# Autodesk Inventor assembly: E-AXIS ASSEMBLY P2.0
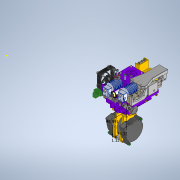
[picture p0: Inventor's stored thumbnail of the model, 180x180]
Saved by Autodesk Inventor 2020.3 (Build 243373010, 373A)
## iProperties
Created: 2019-12-19
Part Number: E-AXIS ASSEMBLY P2.0
Document SubType Name: Assembly
Designer: pepd9
Mass: 917.379 g
Surface Area: 2479.59 cm^2
Volume: 339.663 cm^3
Density: 2.70085 g/cm^3
Author: pepd9
## Documents named in this file (48)
- D:\Designs\MK3PRO P1\E-Axis\E-AXIS ASSEMBLY P2.0.iam
- D:\Designs\MK3PRO P1\E-Axis\X-Carriage V1.3.ipt
- D:\Designs\MK3PRO P1\COMPONENTS\M3 Nut.ipt
- D:\Designs\MK3PRO P1\COMPONENTS\NUT_SQUARE_M3.ipt
- D:\Designs\MK3PRO P1\COMPONENTS\LM10UU.ipt
- D:\Designs\MK3PRO P1\COMPONENTS\SHCS_M3_14.ipt
- D:\Designs\MK3PRO P1\E-Axis\Endstop Trigger Block.ipt
- D:\Designs\MK3PRO P1\COMPONENTS\SHCS_M3_20.ipt
- D:\Designs\MK3PRO P1\E-Axis\Extruder Back V2.ipt
- D:\Designs\MK3PRO P1\COMPONENTS\SHCS_M3_12.ipt
- D:\Designs\MK3PRO P1\E-Axis\Extruder Idler V2.ipt
- D:\Designs\MK3PRO P1\E-Axis\extruder-cover.ipt
- D:\Designs\MK3PRO P1\E-Axis\Fan Support Front.ipt
- D:\Designs\MK3PRO P1\E-Axis\Left Cable Guide.ipt
- D:\Designs\MK3PRO P1\COMPONENTS\SHCS_M3_35.ipt
- D:\Designs\MK3PRO P1\COMPONENTS\SHCS_M3_40.ipt
- D:\Designs\MK3PRO P1\COMPONENTS\Bondtech Idler.ipt
- D:\Designs\MK3PRO P1\E-Axis\PINDA_Probe.ipt
- D:\Designs\MK3PRO P1\E-Axis\E3D_V6.ipt
- D:\Designs\MK3PRO P1\E-Axis\E-Motor Mount P1.1.ipt
- D:\Designs\MK3PRO P1\E-Axis\Extruder_stepper_motor.iam
- D:\Designs\MK3PRO P1\COMPONENTS\SHCS_M3_8.ipt
- D:\Designs\MK3PRO P1\COMPONENTS\Bondtech Driver.ipt
- D:\Designs\MK3PRO P1\COMPONENTS\M3 Washer.ipt
- D:\Designs\MK3PRO P1\COMPONENTS\SHCS_M3_30.ipt
- D:\Designs\MK3PRO P1\COMPONENTS\FAN_5015_BLOWER.ipt
- D:\Designs\MK3PRO P1\COMPONENTS\SHCS_M3_25.ipt
- D:\Designs\MK3PRO P1\E-Axis\x-Carriage Backplate V1.2.ipt
- D:\Designs\MK3PRO P1\COMPONENTS\SHCS_M3_18.ipt
- D:\Designs\MK3PRO P1\E-Axis\LimitSwitch Container.ipt
- D:\Designs\MK3PRO P1\COMPONENTS\Noctua-NF-A4x10.ipt
- D:\Designs\MK3PRO P1\E-Axis\S Fan Cover.ipt
- D:\Designs\MK3PRO P1\COMPONENTS\Small Limit Switch.iam
- D:\Designs\MK3PRO P1\E-Axis\Extruder Cable Clamp.ipt
- D:\Designs\MK3PRO P1\E-Axis\Rear Fan Backplate Mount.ipt
- D:\Designs\MK3PRO P1\E-Axis\Rear Left Fan Mount.ipt
- D:\Designs\MK3PRO P1\E-Axis\Rear Right Fan Mount.ipt
- D:\Designs\MK3PRO P1\E-Axis\Rear Fan Spacer.ipt
- D:\Designs\MK3PRO P1\E2\Solenoid Assembly.iam
- D:\Designs\MK3PRO P1\E2\SolenoidBracket.ipt
- D:\Designs\MK3PRO P1\E2\TW-04-09.iam
- D:\Designs\MK3PRO P1\E2\TS-04-09-100.ipt
- D:\Designs\MK3PRO P1\COMPONENTS\SHCS_M2_10.ipt
- D:\Designs\MK3PRO P1\COMPONENTS\M2 Nut.ipt
- D:\Designs\MK3PRO P1\COMPONENTS\SHCS_M2x8.ipt
- D:\Designs\MK3PRO P1\E2\Slide.ipt
- D:\Designs\MK3PRO P1\E2\Link.ipt
- D:\Designs\MK3PRO P1\E2\extruder-coverE2.ipt
## Components (131 placed, 47 different names)
1. X-Carriage V1.3:1 — Flush:1, Mate:1, Mate:2, Mate:3, Mate:4, Mate:5, Mate:6, Mate:7, Mate:8, Mate:9, Mate:10, Mate:11, Mate:12, Mate:13, Mate:14, Mate:15, Mate:16, Mate:17, Mate:18, Mate:19, Mate:20, Angle:1, Angle:2, Angle:3, Angle:4, Angle:5, Angle:6, Angle:7, Angle:8, Angle:9, Mate:21, Mate:22, Angle:10, Mate:23, Mate:24, Mate:25, Mate:26, Mate:27, Mate:28, Mate:29, Mate:30, Mate:31, Mate:32, Mate:33, Mate:34, Angle:11, Mate:35, Mate:36, Angle:12, Mate:49, Mate:50, Mate:51, Mate:58, Mate:59, Mate:60, Mate:61, Mate:68, Mate:69, Mate:70, Mate:71, Mate:72, Mate:73, Mate:133, Mate:134, Mate:135, Mate:136, Mate:145, Mate:146, Mate:147
2. M3 Nut:1 — Mate:6, Mate:15, Angle:6
3. M3 Nut:2 — Mate:7, Mate:16, Angle:5
4. M3 Nut:3 — Mate:9, Mate:18, Angle:3
5. M3 Nut:4 — Mate:8, Mate:17, Angle:4
6. M3 Nut:5 — Mate:4, Mate:19, Angle:2
7. M3 Nut:6 — Mate:3, Mate:20, Angle:1
8. M3 Nut:7 — Mate:5, Mate:14, Angle:7
9. M3 Nut:8 — Mate:10, Mate:13, Angle:8
10. M3 Nut:9 — Mate:11, Mate:12, Angle:9
11. NUT_SQUARE_M3:1 — Mate:21, Mate:22, Angle:10
12. LM10UU:1 — Mate:25, Mate:28
13. LM10UU:2 — Mate:24, Mate:27
14. LM10UU:3 — Mate:23, Mate:26
15. SHCS_M3_14:1 — Mate:30, Mate:32
16. SHCS_M3_14:2 — Mate:29, Mate:31
17. Endstop Trigger Block:1 — Mate:35, Mate:36, Angle:12, Mate:37, Mate:38
18. NUT_SQUARE_M3:2 — Mate:33, Mate:34, Angle:11
19. SHCS_M3_20:1 — Mate:37, Mate:38
20. Extruder Back V2:1 — Mate:39, Mate:40, Mate:41, Mate:42, Mate:43, Mate:44, Mate:45, Mate:46, Angle:13, Mate:47, Angle:14, Mate:48, Angle:15, Mate:49, Mate:50, Mate:51, Mate:52, Mate:53, Angle:16, Mate:54, Mate:55, Mate:56, Mate:57, Angle:17, Angle:18, Mate:62, Mate:63, Angle:19, Mate:75, Mate:76, Mate:77, Mate:80, Mate:81, Angle:21, Mate:88, Mate:89, Mate:90, Flush:4, Mate:137, Mate:138, Angle:31, Angle:32, Mate:164, Mate:165, Angle:35, Mate:168, Mate:169, Mate:170, Mate:276, Angle:54, Mate:281, Mate:282, Flush:6, Mate:289, Mate:326, Mate:327, Mate:328, Mate:329, Angle:61, Angle:62, Mate:331, Mate:332, Mate:333
21. M3 Nut:10 — Mate:39, Mate:41
22. M3 Nut:11 — Mate:40, Mate:42
23. NUT_SQUARE_M3:3 — Mate:45, Mate:46, Angle:13
24. NUT_SQUARE_M3:4 — Mate:44, Mate:47, Angle:14
25. NUT_SQUARE_M3:5 — Mate:43, Mate:48, Angle:15
26. NUT_SQUARE_M3:6 — Mate:52, Mate:53, Angle:16
27. M3 Nut:12 — Mate:54, Mate:57, Angle:18
28. M3 Nut:13 — Mate:55, Mate:56, Angle:17
29. SHCS_M3_12:1 — Mate:58, Mate:60
30. SHCS_M3_12:2 — Mate:59, Mate:61
31. Extruder Idler V2:1 — Mate:74, Mate:75, Mate:78, Mate:79, Flush:4, Mate:92, Mate:93
32. extruder-cover:1 — Mate:96, Mate:97, Mate:98, Mate:99, Mate:100, Mate:101, Angle:24, Mate:102, Angle:25, Mate:103, Mate:104, Angle:26, Mate:105, Mate:106, Angle:27, Mate:107, Mate:108, Mate:109, Mate:110, Mate:111, Mate:112, Mate:113
33. Fan Support Front:1 — Mate:111, Mate:112, Mate:113, Mate:114, Mate:115, Mate:116, Mate:117, Mate:118, Mate:119, Angle:28, Mate:120, Mate:121, Angle:29, Mate:131, Mate:132, Mate:379, Mate:380
34. Left Cable Guide:1 — Mate:62, Mate:63, Angle:19, Mate:64, Mate:65, Angle:20, Mate:66, Mate:67, Mate:266, Mate:267, Angle:53, Mate:268, Mate:269, Mate:270
35. NUT_SQUARE_M3:7 — Mate:64, Mate:65, Angle:20
36. SHCS_M3_12:3 — Mate:66, Mate:67
37. SHCS_M3_35:1 — Mate:68, Mate:71, Mate:74
38. SHCS_M3_35:2 — Mate:70, Mate:73
39. SHCS_M3_35:3 — Mate:69, Mate:72
40. SHCS_M3_40:1 — Mate:76, Mate:77, Mate:94, Mate:95
41. Bondtech Idler:1 — Mate:78, Mate:79, Flush:3
42. PINDA_Probe:1 — Flush:2
43. E3D_V6:1 — Mate:80, Mate:81, Angle:21, Flush:2, Angle:63
44. E-Motor Mount P1.1:1 — Mate:83, Mate:84, Mate:85, Mate:86, Mate:87, Mate:88, Mate:89, Mate:90, Mate:96, Mate:97, Mate:98
45. Extruder_stepper_motor:1 [sub-assembly] — Mate:83, Mate:84, Mate:85, Mate:91
46. SHCS_M3_8:1 — Mate:86, Mate:87
47. Bondtech Driver:1 — Mate:91, Flush:3
48. M3 Washer:1 — Mate:92, Mate:93
49. M3 Washer:2 — Mate:94, Mate:95
50. NUT_SQUARE_M3:8 — Mate:105, Mate:106, Angle:27
51. NUT_SQUARE_M3:9 — Mate:103, Mate:104, Angle:26
52. NUT_SQUARE_M3:10 — Mate:100, Mate:101, Angle:24
53. NUT_SQUARE_M3:11 — Mate:99, Mate:102, Angle:25
54. SHCS_M3_30:1 — Mate:107, Mate:108
55. SHCS_M3_30:2 — Mate:109, Mate:110
56. M3 Nut:14 — Mate:118, Mate:119, Angle:28
57. M3 Nut:15 — Mate:120, Mate:121, Angle:29
58. SHCS_M3_8:2 — Mate:114, Mate:117
59. SHCS_M3_8:3 — Mate:115, Mate:116
60. SHCS_M3_20:2 — Mate:129, Mate:130, Mate:383
61. M3 Washer:3 — Mate:129, Mate:130, Mate:382
62. SHCS_M3_25:1 — Mate:131, Mate:132, Mate:381
63. SHCS_M3_12:4 — Mate:133, Mate:136, Mate:140
64. SHCS_M3_12:5 — Mate:134, Mate:135, Mate:139
65. M3 Nut:16 — Mate:137, Mate:140, Angle:32
66. M3 Nut:17 — Mate:138, Mate:139, Angle:31
67. x-Carriage Backplate V1.2:1 — Mate:141, Mate:142, Mate:143, Mate:144, Angle:33, Angle:34, Mate:145, Mate:146, Mate:147, Mate:148, Mate:149, Mate:150, Mate:151, Mate:152, Mate:153, Mate:154, Mate:155, Mate:156, Mate:157, Mate:158, Mate:159, Mate:160, Mate:161, Mate:162, Mate:163, Mate:187, Mate:214, Mate:275
68. M3 Nut:18 — Mate:141, Mate:144, Angle:33
69. M3 Nut:19 — Mate:142, Mate:143, Angle:34
70. SHCS_M3_18:1 — Mate:148, Mate:153
71. SHCS_M3_18:2 — Mate:149, Mate:151
72. SHCS_M3_18:3 — Mate:150, Mate:152
73. SHCS_M3_18:4 — Mate:154, Mate:155
74. SHCS_M3_18:5 — Mate:156, Mate:158
75. SHCS_M3_18:6 — Mate:157, Mate:159
76. SHCS_M3_18:7 — Mate:160, Mate:163
77. SHCS_M3_18:8 — Mate:161, Mate:162
78. LimitSwitch Container:1 — Mate:164, Mate:165, Angle:35, Mate:166, Mate:167, Mate:179, Mate:180, Mate:181
79. SHCS_M3_8:4 — Mate:166, Mate:167
80. Noctua-NF-A4x10:1 — Mate:168, Mate:169, Mate:170, Mate:171, Mate:172, Mate:173, Mate:174, Mate:248
81. SHCS_M3_18:9 — Mate:172, Mate:249
82. SHCS_M3_18:10 — Mate:171
83. SHCS_M3_18:11 — Mate:173, Mate:250
84. SHCS_M3_18:12 — Mate:174
85. Small Limit Switch:1 [sub-assembly] — Mate:179, Mate:180, Mate:181
86. Rear Fan Backplate Mount:1 — Mate:182, Mate:183, Mate:184, Mate:185, Angle:37, Mate:187, Mate:188, Mate:189, Mate:190, Mate:191, Mate:200, Mate:201, Mate:202, Mate:203, Angle:52, Mate:275
87. M3 Nut:20 — Mate:182, Mate:184
88. M3 Nut:21 — Mate:183, Mate:185, Angle:37
89. SHCS_M3_12:6 — Mate:188, Mate:189
90. SHCS_M3_14:3 — Mate:190, Mate:191, Mate:214
91. Rear Left Fan Mount:1 — Mate:198, Angle:40, Mate:201, Mate:202, Mate:205, Mate:206, Mate:207, Mate:219, Mate:222, Angle:52, Mate:374, Angle:66
92. Rear Right Fan Mount:1 — Mate:196, Angle:42, Mate:200, Mate:203, Mate:204, Mate:208, Mate:209, Mate:220, Mate:221, Mate:373, Angle:65, Mate:377
93. M3 Nut:22 — Mate:196, Angle:42, Mate:265
94. M3 Nut:25 — Mate:198, Angle:40, Mate:246
95. FAN_5015_BLOWER:2 — Mate:204, Mate:208, Mate:209, Mate:242, Mate:243, Mate:255, Mate:256
96. FAN_5015_BLOWER:3 — Mate:205, Mate:206, Mate:207, Mate:240, Mate:241, Mate:371, Mate:372
97. SHCS_M3_14:4 — Mate:219, Mate:222
98. SHCS_M3_14:5 — Mate:220, Mate:221
99. SHCS_M3_25:2 — Mate:240, Mate:241, Mate:247
100. SHCS_M3_25:3 — Mate:242, Mate:244, Mate:245
101. M3 Washer:4 — Mate:243, Mate:244, Mate:245
102. Rear Fan Spacer:1 — Mate:246, Mate:247, Mate:265
103. S Fan Cover:1 — Mate:248, Mate:249, Mate:250
104. SHCS_M3_18:13 — Mate:271, Mate:274
105. SHCS_M3_25:4 — Mate:255, Mate:257, Mate:258, Mate:376, Mate:378
106. M3 Washer:5 — Mate:256, Mate:257, Mate:258
107. NUT_SQUARE_M3:12 — Mate:266, Mate:267, Angle:53
108. SHCS_M3_18:14 — Mate:272, Mate:273
109. Extruder Cable Clamp:1 — Mate:268, Mate:269, Mate:270, Mate:271, Mate:272, Mate:273, Mate:274
110. Solenoid Assembly:1 [sub-assembly] — Mate:276, Angle:54, Mate:278, Mate:280
111. SolenoidBracket:1 — Mate:278, Mate:280, Mate:281, Mate:282
112. TW-04-09:1 [sub-assembly] — Mate:290, Mate:300, Mate:341, Mate:342, Mate:361
113. TS-04-09-100:1 — Mate:289, Mate:290, Flush:6, Mate:300
114. SHCS_M2_10:1 — Flush:15
115. SHCS_M2_10:3 — Flush:13, Mate:342, Mate:362
116. SHCS_M2_10:4 — Flush:13, Flush:14, Flush:15
117. M2 Nut:1 — Mate:326, Mate:329, Angle:61
118. M2 Nut:2 — Mate:327, Mate:328, Angle:62
119. SHCS_M2x8:2 — Mate:331, Flush:12
120. SHCS_M2x8:3 — Mate:332, Mate:333, Flush:12
121. SHCS_M2_10:5 — Flush:14, Mate:341, Mate:363
122. extruder-coverE2:1 — Mate:365, Angle:64, Mate:367
123. Link:1 — Mate:358, Mate:359, Mate:360
124. Slide:1 — Mate:358, Mate:359, Mate:360, Mate:361, Mate:362, Mate:363, Mate:364, Flush:16, Angle:64, Mate:368, Mate:369, Mate:370
125. E3D_V6:2 — Mate:364, Flush:16, Angle:63, Mate:365
126. Noctua-NF-A4x10:2 — Mate:367, Mate:368, Mate:369, Mate:370
127. SHCS_M3_25:5 — Mate:371, Mate:372, Mate:375
128. M3 Nut:26 — Mate:373, Mate:376, Angle:65
129. M3 Nut:27 — Mate:374, Mate:375, Angle:66
130. Rear Fan Spacer:2 — Mate:377, Mate:378
131. FAN_5015_BLOWER:4 — Mate:379, Mate:380, Mate:381, Mate:382, Mate:383
## Relationships (317: Mate 263, Angle 44, Flush 10)
- Flush:1: X-Carriage V1.3:1
- Mate:1 (8.3 mm): X-Carriage V1.3:1
- Mate:2 (-43.75 mm): X-Carriage V1.3:1
- Mate:3: X-Carriage V1.3:1 ↔ M3 Nut:6
- Mate:4: X-Carriage V1.3:1 ↔ M3 Nut:5
- Mate:5: X-Carriage V1.3:1 ↔ M3 Nut:7
- Mate:6: X-Carriage V1.3:1 ↔ M3 Nut:1
- Mate:7: X-Carriage V1.3:1 ↔ M3 Nut:2
- Mate:8: X-Carriage V1.3:1 ↔ M3 Nut:4
- Mate:9: X-Carriage V1.3:1 ↔ M3 Nut:3
- Mate:10: X-Carriage V1.3:1 ↔ M3 Nut:8
- Mate:11: X-Carriage V1.3:1 ↔ M3 Nut:9
- Mate:12: X-Carriage V1.3:1 ↔ M3 Nut:9
- Mate:13: X-Carriage V1.3:1 ↔ M3 Nut:8
- Mate:14: X-Carriage V1.3:1 ↔ M3 Nut:7
- Mate:15: X-Carriage V1.3:1 ↔ M3 Nut:1
- Mate:16: X-Carriage V1.3:1 ↔ M3 Nut:2
- Mate:17: X-Carriage V1.3:1 ↔ M3 Nut:4
- Mate:18: X-Carriage V1.3:1 ↔ M3 Nut:3
- Mate:19: X-Carriage V1.3:1 ↔ M3 Nut:5
- Mate:20: X-Carriage V1.3:1 ↔ M3 Nut:6
- Angle:1 (0 deg): X-Carriage V1.3:1 ↔ M3 Nut:6
- Angle:2 (0 deg): X-Carriage V1.3:1 ↔ M3 Nut:5
- Angle:3 (0 deg): X-Carriage V1.3:1 ↔ M3 Nut:3
- Angle:4 (0 deg): X-Carriage V1.3:1 ↔ M3 Nut:4
- Angle:5 (0 deg): X-Carriage V1.3:1 ↔ M3 Nut:2
- Angle:6 (0 deg): X-Carriage V1.3:1 ↔ M3 Nut:1
- Angle:7 (0 deg): X-Carriage V1.3:1 ↔ M3 Nut:7
- Angle:8 (0 deg): X-Carriage V1.3:1 ↔ M3 Nut:8
- Angle:9 (0 deg): X-Carriage V1.3:1 ↔ M3 Nut:9
- Mate:21: X-Carriage V1.3:1 ↔ NUT_SQUARE_M3:1
- Mate:22: X-Carriage V1.3:1 ↔ NUT_SQUARE_M3:1
- Angle:10 (0 deg): X-Carriage V1.3:1 ↔ NUT_SQUARE_M3:1
- Mate:23: X-Carriage V1.3:1 ↔ LM10UU:3
- Mate:24: X-Carriage V1.3:1 ↔ LM10UU:2
- Mate:25: X-Carriage V1.3:1 ↔ LM10UU:1
- Mate:26 (0.25 mm): X-Carriage V1.3:1 ↔ LM10UU:3
- Mate:27 (0.25 mm): X-Carriage V1.3:1 ↔ LM10UU:2
- Mate:28 (0.25 mm): X-Carriage V1.3:1 ↔ LM10UU:1
- Mate:29: X-Carriage V1.3:1 ↔ SHCS_M3_14:2
- Mate:30: X-Carriage V1.3:1 ↔ SHCS_M3_14:1
- Mate:31: X-Carriage V1.3:1 ↔ SHCS_M3_14:2
- Mate:32: X-Carriage V1.3:1 ↔ SHCS_M3_14:1
- Mate:33: X-Carriage V1.3:1 ↔ NUT_SQUARE_M3:2
- Mate:34: X-Carriage V1.3:1 ↔ NUT_SQUARE_M3:2
- Angle:11 (0 deg): X-Carriage V1.3:1 ↔ NUT_SQUARE_M3:2
- Mate:35: X-Carriage V1.3:1 ↔ Endstop Trigger Block:1
- Mate:36: X-Carriage V1.3:1 ↔ Endstop Trigger Block:1
- Angle:12 (180 deg): X-Carriage V1.3:1 ↔ Endstop Trigger Block:1
- Mate:37: Endstop Trigger Block:1 ↔ SHCS_M3_20:1
- Mate:38: Endstop Trigger Block:1 ↔ SHCS_M3_20:1
- Mate:39: Extruder Back V2:1 ↔ M3 Nut:10
- Mate:40: Extruder Back V2:1 ↔ M3 Nut:11
- Mate:41: Extruder Back V2:1 ↔ M3 Nut:10
- Mate:42: Extruder Back V2:1 ↔ M3 Nut:11
- Mate:43: Extruder Back V2:1 ↔ NUT_SQUARE_M3:5
- Mate:44: Extruder Back V2:1 ↔ NUT_SQUARE_M3:4
- Mate:45: Extruder Back V2:1 ↔ NUT_SQUARE_M3:3
- Mate:46: Extruder Back V2:1 ↔ NUT_SQUARE_M3:3
- Angle:13 (0 deg): Extruder Back V2:1 ↔ NUT_SQUARE_M3:3
- Mate:47: Extruder Back V2:1 ↔ NUT_SQUARE_M3:4
- Angle:14 (0 deg): Extruder Back V2:1 ↔ NUT_SQUARE_M3:4
- Mate:48: Extruder Back V2:1 ↔ NUT_SQUARE_M3:5
- Angle:15 (0 deg): Extruder Back V2:1 ↔ NUT_SQUARE_M3:5
- Mate:49: X-Carriage V1.3:1 ↔ Extruder Back V2:1
- Mate:50: X-Carriage V1.3:1 ↔ Extruder Back V2:1
- Mate:51: X-Carriage V1.3:1 ↔ Extruder Back V2:1
- Mate:52: Extruder Back V2:1 ↔ NUT_SQUARE_M3:6
- Mate:53: Extruder Back V2:1 ↔ NUT_SQUARE_M3:6
- Angle:16 (0 deg): Extruder Back V2:1 ↔ NUT_SQUARE_M3:6
- Mate:54: Extruder Back V2:1 ↔ M3 Nut:12
- Mate:55: Extruder Back V2:1 ↔ M3 Nut:13
- Mate:56: Extruder Back V2:1 ↔ M3 Nut:13
- Mate:57: Extruder Back V2:1 ↔ M3 Nut:12
- Angle:17 (0 deg): Extruder Back V2:1 ↔ M3 Nut:13
- Angle:18 (0 deg): Extruder Back V2:1 ↔ M3 Nut:12
- Mate:58: X-Carriage V1.3:1 ↔ SHCS_M3_12:1
- Mate:59: X-Carriage V1.3:1 ↔ SHCS_M3_12:2
- Mate:60: X-Carriage V1.3:1 ↔ SHCS_M3_12:1
- Mate:61: X-Carriage V1.3:1 ↔ SHCS_M3_12:2
- Mate:62: Extruder Back V2:1 ↔ Left Cable Guide:1
- Mate:63: Extruder Back V2:1 ↔ Left Cable Guide:1
- Angle:19 (180 deg): Extruder Back V2:1 ↔ Left Cable Guide:1
- Mate:64: Left Cable Guide:1 ↔ NUT_SQUARE_M3:7
- Mate:65: Left Cable Guide:1 ↔ NUT_SQUARE_M3:7
- Angle:20 (0 deg): Left Cable Guide:1 ↔ NUT_SQUARE_M3:7
- Mate:66: Left Cable Guide:1 ↔ SHCS_M3_12:3
- Mate:67: Left Cable Guide:1 ↔ SHCS_M3_12:3
- Mate:68: X-Carriage V1.3:1 ↔ SHCS_M3_35:1
- Mate:69: X-Carriage V1.3:1 ↔ SHCS_M3_35:3
- Mate:70: X-Carriage V1.3:1 ↔ SHCS_M3_35:2
- Mate:71: X-Carriage V1.3:1 ↔ SHCS_M3_35:1
- Mate:72: X-Carriage V1.3:1 ↔ SHCS_M3_35:3
- Mate:73: X-Carriage V1.3:1 ↔ SHCS_M3_35:2
- Mate:74: Extruder Idler V2:1 ↔ SHCS_M3_35:1
- Mate:75 (0.5 mm): Extruder Back V2:1 ↔ Extruder Idler V2:1
- Mate:76: Extruder Back V2:1 ↔ SHCS_M3_40:1
- Mate:77: Extruder Back V2:1 ↔ SHCS_M3_40:1
- Mate:78: Extruder Idler V2:1 ↔ Bondtech Idler:1
- Mate:79 (0.25 mm): Extruder Idler V2:1 ↔ Bondtech Idler:1
- Mate:80: Extruder Back V2:1 ↔ E3D_V6:1
- Mate:81: Extruder Back V2:1 ↔ E3D_V6:1
- Angle:21 (90 deg): Extruder Back V2:1 ↔ E3D_V6:1
- Flush:2 (2 mm): PINDA_Probe:1 ↔ E3D_V6:1
- Mate:83: E-Motor Mount P1.1:1 ↔ Extruder_stepper_motor:1
- Mate:84: E-Motor Mount P1.1:1 ↔ Extruder_stepper_motor:1
- Mate:85: E-Motor Mount P1.1:1 ↔ Extruder_stepper_motor:1
- Mate:86: E-Motor Mount P1.1:1 ↔ SHCS_M3_8:1
- Mate:87: E-Motor Mount P1.1:1 ↔ SHCS_M3_8:1
- Mate:88: Extruder Back V2:1 ↔ E-Motor Mount P1.1:1
- Mate:89: Extruder Back V2:1 ↔ E-Motor Mount P1.1:1
- Mate:90: Extruder Back V2:1 ↔ E-Motor Mount P1.1:1
- Mate:91: Extruder_stepper_motor:1 ↔ Bondtech Driver:1
- Flush:3: Bondtech Idler:1 ↔ Bondtech Driver:1
- Flush:4: Extruder Back V2:1 ↔ Extruder Idler V2:1
- Mate:92: Extruder Idler V2:1 ↔ M3 Washer:1
- Mate:93: Extruder Idler V2:1 ↔ M3 Washer:1
- Mate:94: SHCS_M3_40:1 ↔ M3 Washer:2
- Mate:95: SHCS_M3_40:1 ↔ M3 Washer:2
- Mate:96: extruder-cover:1 ↔ E-Motor Mount P1.1:1
- Mate:97: extruder-cover:1 ↔ E-Motor Mount P1.1:1
- Mate:98: extruder-cover:1 ↔ E-Motor Mount P1.1:1
- Mate:99: extruder-cover:1 ↔ NUT_SQUARE_M3:11
- Mate:100: extruder-cover:1 ↔ NUT_SQUARE_M3:10
- Mate:101: extruder-cover:1 ↔ NUT_SQUARE_M3:10
- Angle:24 (0 deg): extruder-cover:1 ↔ NUT_SQUARE_M3:10
- Mate:102: extruder-cover:1 ↔ NUT_SQUARE_M3:11
- Angle:25 (0 deg): extruder-cover:1 ↔ NUT_SQUARE_M3:11
- Mate:103: extruder-cover:1 ↔ NUT_SQUARE_M3:9
- Mate:104: extruder-cover:1 ↔ NUT_SQUARE_M3:9
- Angle:26 (0 deg): extruder-cover:1 ↔ NUT_SQUARE_M3:9
- Mate:105: extruder-cover:1 ↔ NUT_SQUARE_M3:8
- Mate:106: extruder-cover:1 ↔ NUT_SQUARE_M3:8
- Angle:27 (0 deg): extruder-cover:1 ↔ NUT_SQUARE_M3:8
- Mate:107: extruder-cover:1 ↔ SHCS_M3_30:1
- Mate:108: extruder-cover:1 ↔ SHCS_M3_30:1
- Mate:109: extruder-cover:1 ↔ SHCS_M3_30:2
- Mate:110: extruder-cover:1 ↔ SHCS_M3_30:2
- Mate:111: extruder-cover:1 ↔ Fan Support Front:1
- Mate:112: extruder-cover:1 ↔ Fan Support Front:1
- Mate:113: extruder-cover:1 ↔ Fan Support Front:1
- Mate:114: Fan Support Front:1 ↔ SHCS_M3_8:2
- Mate:115: Fan Support Front:1 ↔ SHCS_M3_8:3
- Mate:116: Fan Support Front:1 ↔ SHCS_M3_8:3
- Mate:117: Fan Support Front:1 ↔ SHCS_M3_8:2
- Mate:118: Fan Support Front:1 ↔ M3 Nut:14
- Mate:119: Fan Support Front:1 ↔ M3 Nut:14
- Angle:28 (0 deg): Fan Support Front:1 ↔ M3 Nut:14
- Mate:120: Fan Support Front:1 ↔ M3 Nut:15
- Mate:121: Fan Support Front:1 ↔ M3 Nut:15
- Angle:29 (30 deg): Fan Support Front:1 ↔ M3 Nut:15
- Mate:129: SHCS_M3_20:2 ↔ M3 Washer:3
- Mate:130: SHCS_M3_20:2 ↔ M3 Washer:3
- Mate:131: Fan Support Front:1 ↔ SHCS_M3_25:1
- Mate:132: Fan Support Front:1 ↔ SHCS_M3_25:1
- Mate:133: X-Carriage V1.3:1 ↔ SHCS_M3_12:4
- Mate:134: X-Carriage V1.3:1 ↔ SHCS_M3_12:5
- Mate:135: X-Carriage V1.3:1 ↔ SHCS_M3_12:5
- Mate:136: X-Carriage V1.3:1 ↔ SHCS_M3_12:4
- Mate:137: Extruder Back V2:1 ↔ M3 Nut:16
- Mate:138: Extruder Back V2:1 ↔ M3 Nut:17
- Mate:139: SHCS_M3_12:5 ↔ M3 Nut:17
- Angle:31 (0 deg): Extruder Back V2:1 ↔ M3 Nut:17
- Mate:140: SHCS_M3_12:4 ↔ M3 Nut:16
- Angle:32 (0 deg): Extruder Back V2:1 ↔ M3 Nut:16
- Mate:141: x-Carriage Backplate V1.2:1 ↔ M3 Nut:18
- Mate:142: x-Carriage Backplate V1.2:1 ↔ M3 Nut:19
- Mate:143: x-Carriage Backplate V1.2:1 ↔ M3 Nut:19
- Mate:144: x-Carriage Backplate V1.2:1 ↔ M3 Nut:18
- Angle:33 (0 deg): x-Carriage Backplate V1.2:1 ↔ M3 Nut:18
- Angle:34 (0 deg): x-Carriage Backplate V1.2:1 ↔ M3 Nut:19
- Mate:145: X-Carriage V1.3:1 ↔ x-Carriage Backplate V1.2:1
- Mate:146: X-Carriage V1.3:1 ↔ x-Carriage Backplate V1.2:1
- Mate:147: X-Carriage V1.3:1 ↔ x-Carriage Backplate V1.2:1
- Mate:148: x-Carriage Backplate V1.2:1 ↔ SHCS_M3_18:1
- Mate:149: x-Carriage Backplate V1.2:1 ↔ SHCS_M3_18:2
- Mate:150: x-Carriage Backplate V1.2:1 ↔ SHCS_M3_18:3
- Mate:151: x-Carriage Backplate V1.2:1 ↔ SHCS_M3_18:2
- Mate:152: x-Carriage Backplate V1.2:1 ↔ SHCS_M3_18:3
- Mate:153: x-Carriage Backplate V1.2:1 ↔ SHCS_M3_18:1
- Mate:154: x-Carriage Backplate V1.2:1 ↔ SHCS_M3_18:4
- Mate:155: x-Carriage Backplate V1.2:1 ↔ SHCS_M3_18:4
- Mate:156: x-Carriage Backplate V1.2:1 ↔ SHCS_M3_18:5
- Mate:157: x-Carriage Backplate V1.2:1 ↔ SHCS_M3_18:6
- Mate:158: x-Carriage Backplate V1.2:1 ↔ SHCS_M3_18:5
- Mate:159: x-Carriage Backplate V1.2:1 ↔ SHCS_M3_18:6
- Mate:160: x-Carriage Backplate V1.2:1 ↔ SHCS_M3_18:7
- Mate:161: x-Carriage Backplate V1.2:1 ↔ SHCS_M3_18:8
- Mate:162: x-Carriage Backplate V1.2:1 ↔ SHCS_M3_18:8
- Mate:163: x-Carriage Backplate V1.2:1 ↔ SHCS_M3_18:7
- Mate:164: Extruder Back V2:1 ↔ LimitSwitch Container:1
- Mate:165: Extruder Back V2:1 ↔ LimitSwitch Container:1
- Angle:35 (180 deg): Extruder Back V2:1 ↔ LimitSwitch Container:1
- Mate:166: LimitSwitch Container:1 ↔ SHCS_M3_8:4
- Mate:167: LimitSwitch Container:1 ↔ SHCS_M3_8:4
- Mate:168: Extruder Back V2:1 ↔ Noctua-NF-A4x10:1
- Mate:169: Extruder Back V2:1 ↔ Noctua-NF-A4x10:1
- Mate:170: Extruder Back V2:1 ↔ Noctua-NF-A4x10:1
- Mate:171: Noctua-NF-A4x10:1 ↔ SHCS_M3_18:10
- Mate:172: Noctua-NF-A4x10:1 ↔ SHCS_M3_18:9
- Mate:173: Noctua-NF-A4x10:1 ↔ SHCS_M3_18:11
- Mate:174: Noctua-NF-A4x10:1 ↔ SHCS_M3_18:12
- Mate:179: LimitSwitch Container:1 ↔ Small Limit Switch:1
- Mate:180: LimitSwitch Container:1 ↔ Small Limit Switch:1
- Mate:181: LimitSwitch Container:1 ↔ Small Limit Switch:1
- Mate:182: Rear Fan Backplate Mount:1 ↔ M3 Nut:20
- Mate:183: Rear Fan Backplate Mount:1 ↔ M3 Nut:21
- Mate:184: Rear Fan Backplate Mount:1 ↔ M3 Nut:20
- Mate:185: Rear Fan Backplate Mount:1 ↔ M3 Nut:21
- Angle:37 (0 deg): Rear Fan Backplate Mount:1 ↔ M3 Nut:21
- Mate:187: x-Carriage Backplate V1.2:1 ↔ Rear Fan Backplate Mount:1
- Mate:188: Rear Fan Backplate Mount:1 ↔ SHCS_M3_12:6
- Mate:189: Rear Fan Backplate Mount:1 ↔ SHCS_M3_12:6
- Mate:190: Rear Fan Backplate Mount:1 ↔ SHCS_M3_14:3
- Mate:191: Rear Fan Backplate Mount:1 ↔ SHCS_M3_14:3
- Mate:196: Rear Right Fan Mount:1 ↔ M3 Nut:22
- Mate:198: Rear Left Fan Mount:1 ↔ M3 Nut:25
- Angle:40 (0 deg): Rear Left Fan Mount:1 ↔ M3 Nut:25
- Angle:42 (0 deg): Rear Right Fan Mount:1 ↔ M3 Nut:22
- Mate:200: Rear Fan Backplate Mount:1 ↔ Rear Right Fan Mount:1
- Mate:201: Rear Fan Backplate Mount:1 ↔ Rear Left Fan Mount:1
- Mate:202: Rear Fan Backplate Mount:1 ↔ Rear Left Fan Mount:1
- Mate:203: Rear Fan Backplate Mount:1 ↔ Rear Right Fan Mount:1
- Mate:204: Rear Right Fan Mount:1 ↔ FAN_5015_BLOWER:2
- Mate:205: Rear Left Fan Mount:1 ↔ FAN_5015_BLOWER:3
- Mate:206: Rear Left Fan Mount:1 ↔ FAN_5015_BLOWER:3
- Mate:207: Rear Left Fan Mount:1 ↔ FAN_5015_BLOWER:3
- Mate:208: Rear Right Fan Mount:1 ↔ FAN_5015_BLOWER:2
- Mate:209: Rear Right Fan Mount:1 ↔ FAN_5015_BLOWER:2
- Mate:214: x-Carriage Backplate V1.2:1 ↔ SHCS_M3_14:3
- Mate:219: Rear Left Fan Mount:1 ↔ SHCS_M3_14:4
- Mate:220: Rear Right Fan Mount:1 ↔ SHCS_M3_14:5
- Mate:221: Rear Right Fan Mount:1 ↔ SHCS_M3_14:5
- Mate:222: Rear Left Fan Mount:1 ↔ SHCS_M3_14:4
- Mate:240: FAN_5015_BLOWER:3 ↔ SHCS_M3_25:2
- Mate:241: FAN_5015_BLOWER:3 ↔ SHCS_M3_25:2
- Mate:242: FAN_5015_BLOWER:2 ↔ SHCS_M3_25:3
- Mate:243: FAN_5015_BLOWER:2 ↔ M3 Washer:4
- Mate:244: SHCS_M3_25:3 ↔ M3 Washer:4
- Mate:245: SHCS_M3_25:3 ↔ M3 Washer:4
- Mate:246: M3 Nut:25 ↔ Rear Fan Spacer:1
- Mate:247: SHCS_M3_25:2 ↔ Rear Fan Spacer:1
- Mate:248: Noctua-NF-A4x10:1 ↔ S Fan Cover:1
- Mate:249: SHCS_M3_18:9 ↔ S Fan Cover:1
- Mate:250: SHCS_M3_18:11 ↔ S Fan Cover:1
- Mate:255: FAN_5015_BLOWER:2 ↔ SHCS_M3_25:4
- Mate:256: FAN_5015_BLOWER:2 ↔ M3 Washer:5
- Mate:257: SHCS_M3_25:4 ↔ M3 Washer:5
- Mate:258: SHCS_M3_25:4 ↔ M3 Washer:5
- Mate:265: M3 Nut:22 ↔ Rear Fan Spacer:1
- Angle:52 (0 deg): Rear Fan Backplate Mount:1 ↔ Rear Left Fan Mount:1
- Mate:266: Left Cable Guide:1 ↔ NUT_SQUARE_M3:12
- Mate:267: Left Cable Guide:1 ↔ NUT_SQUARE_M3:12
- Angle:53 (0 deg): Left Cable Guide:1 ↔ NUT_SQUARE_M3:12
- Mate:268: Left Cable Guide:1 ↔ Extruder Cable Clamp:1
- Mate:269: Left Cable Guide:1 ↔ Extruder Cable Clamp:1
- Mate:270: Left Cable Guide:1 ↔ Extruder Cable Clamp:1
- Mate:271: SHCS_M3_18:13 ↔ Extruder Cable Clamp:1
- Mate:272: SHCS_M3_18:14 ↔ Extruder Cable Clamp:1
- Mate:273: SHCS_M3_18:14 ↔ Extruder Cable Clamp:1
- Mate:274: SHCS_M3_18:13 ↔ Extruder Cable Clamp:1
- Mate:275: x-Carriage Backplate V1.2:1 ↔ Rear Fan Backplate Mount:1
- Mate:276: Extruder Back V2:1 ↔ Solenoid Assembly:1
- Angle:54 (0 deg): Extruder Back V2:1 ↔ Solenoid Assembly:1
- Mate:278: Solenoid Assembly:1 ↔ SolenoidBracket:1
- Mate:280: Solenoid Assembly:1 ↔ SolenoidBracket:1
- Mate:281: Extruder Back V2:1 ↔ SolenoidBracket:1
- Mate:282: Extruder Back V2:1 ↔ SolenoidBracket:1
- Mate:289: Extruder Back V2:1 ↔ TS-04-09-100:1
- Mate:290: TW-04-09:1 ↔ TS-04-09-100:1
- Flush:6: Extruder Back V2:1 ↔ TS-04-09-100:1
- Mate:300: TW-04-09:1 ↔ TS-04-09-100:1
- Mate:326: Extruder Back V2:1 ↔ M2 Nut:1
- Mate:327: Extruder Back V2:1 ↔ M2 Nut:2
- Mate:328: Extruder Back V2:1 ↔ M2 Nut:2
- Mate:329: Extruder Back V2:1 ↔ M2 Nut:1
- Angle:61 (0 deg): Extruder Back V2:1 ↔ M2 Nut:1
- Angle:62 (0 deg): Extruder Back V2:1 ↔ M2 Nut:2
- Mate:331: Extruder Back V2:1 ↔ SHCS_M2x8:2
- Mate:332: Extruder Back V2:1 ↔ SHCS_M2x8:3
- Mate:333 (4.6 mm): Extruder Back V2:1 ↔ SHCS_M2x8:3
- Flush:12: SHCS_M2x8:2 ↔ SHCS_M2x8:3
- Flush:13: SHCS_M2_10:3 ↔ SHCS_M2_10:4
- Flush:14: SHCS_M2_10:4 ↔ SHCS_M2_10:5
- Flush:15: SHCS_M2_10:1 ↔ SHCS_M2_10:4
- Mate:341: TW-04-09:1 ↔ SHCS_M2_10:5
- Mate:342: TW-04-09:1 ↔ SHCS_M2_10:3
- Mate:358: Link:1 ↔ Slide:1
- Mate:359: Link:1 ↔ Slide:1
- Mate:360: Link:1 ↔ Slide:1
- Mate:361: TW-04-09:1 ↔ Slide:1
- Mate:362: SHCS_M2_10:3 ↔ Slide:1
- Mate:363: SHCS_M2_10:5 ↔ Slide:1
- Mate:364: Slide:1 ↔ E3D_V6:2
- Flush:16: Slide:1 ↔ E3D_V6:2
- Angle:63 (0 deg): E3D_V6:1 ↔ E3D_V6:2
- Mate:365: extruder-coverE2:1 ↔ E3D_V6:2
- Angle:64 (0 deg): extruder-coverE2:1 ↔ Slide:1
- Mate:367: extruder-coverE2:1 ↔ Noctua-NF-A4x10:2
- Mate:368: Slide:1 ↔ Noctua-NF-A4x10:2
- Mate:369: Slide:1 ↔ Noctua-NF-A4x10:2
- Mate:370: Slide:1 ↔ Noctua-NF-A4x10:2
- Mate:371: FAN_5015_BLOWER:3 ↔ SHCS_M3_25:5
- Mate:372: FAN_5015_BLOWER:3 ↔ SHCS_M3_25:5
- Mate:373: Rear Right Fan Mount:1 ↔ M3 Nut:26
- Mate:374: Rear Left Fan Mount:1 ↔ M3 Nut:27
- Mate:375: SHCS_M3_25:5 ↔ M3 Nut:27
- Mate:376: SHCS_M3_25:4 ↔ M3 Nut:26
- Angle:65 (0 deg): Rear Right Fan Mount:1 ↔ M3 Nut:26
- Angle:66 (0 deg): Rear Left Fan Mount:1 ↔ M3 Nut:27
- Mate:377: Rear Right Fan Mount:1 ↔ Rear Fan Spacer:2
- Mate:378: SHCS_M3_25:4 ↔ Rear Fan Spacer:2
- Mate:379: Fan Support Front:1 ↔ FAN_5015_BLOWER:4
- Mate:380: Fan Support Front:1 ↔ FAN_5015_BLOWER:4
- Mate:381: SHCS_M3_25:1 ↔ FAN_5015_BLOWER:4
- Mate:382: M3 Washer:3 ↔ FAN_5015_BLOWER:4
- Mate:383: SHCS_M3_20:2 ↔ FAN_5015_BLOWER:4
